# Autodesk Inventor assembly: sense3
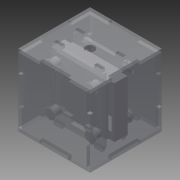
[picture p0: Inventor's stored thumbnail of the model, 180x180]
Saved by Autodesk Inventor 2013 (Build 170138000, 138)
## iProperties
Created: 2014-05-23
Part Number: sense3
Document SubType Name: Assembly
Designer: balogh
Author: balogh
## Documents named in this file (9)
- C:\Users\Brett Ian Balogh\Documents\GitHub\sense_cube\sense3_inventor\sense3.iam
- C:\Users\Brett Ian Balogh\Documents\GitHub\sense_cube\sense3_inventor\inside_box_top_bot.ipt
- C:\Users\Brett Ian Balogh\Documents\GitHub\sense_cube\sense3_inventor\pcb_mount.ipt
- C:\Users\Brett Ian Balogh\Documents\GitHub\sense_cube\sense3_inventor\battery_mount.ipt
- C:\Users\Brett Ian Balogh\Documents\GitHub\sense_cube\sense3_inventor\pcb.ipt
- C:\Users\Brett Ian Balogh\Documents\GitHub\sense_cube\sense3_inventor\inside_box_front_back.ipt
- C:\Users\Brett Ian Balogh\Documents\GitHub\sense_cube\sense3_inventor\inside_box_left_right.ipt
- C:\Users\Brett Ian Balogh\Documents\GitHub\sense_cube\sense3_inventor\thumbscrew_6-32x1.ipt
- C:\Users\Brett Ian Balogh\Documents\GitHub\sense_cube\sense3_inventor\thumbnut_6-32.ipt
## Components (22 placed, 8 different names)
1. inside_box_top_bot:1 — Angle:1, Mate:1, Mate:2, Mate:3, Mate:4, Flush:3, Flush:4, Mate:17, Mate:21, Mate:22
2. inside_box_top_bot:2 — Mate:5, Mate:6, Flush:1, Flush:2, Mate:13, Flush:5, Mate:14, Mate:15, Flush:6, Mate:16, Mate:20, Flush:7
3. pcb_mount:1 — Mate:3, Mate:4, Flush:2, Flush:4, Insert:21, Insert:22, Insert:23, Insert:24
4. pcb_mount:2 — Angle:1, Mate:1, Mate:2, Mate:5, Mate:6, Flush:1, Mate:12, Flush:3, Insert:17, Insert:18, Insert:19, Insert:20
5. battery_mount:1 — Insert:7, Insert:8, Insert:9, Insert:10
6. battery_mount:2 — Insert:9, Insert:10, Insert:11, Insert:12
7. battery_mount:3 — Insert:11, Insert:12, Insert:13, Insert:14
8. battery_mount:4 — Insert:13, Insert:14, Insert:15, Insert:16
9. pcb:1 — Insert:15, Insert:16
10. pcb:2 — Insert:7, Insert:8, Mate:12
11. inside_box_front_back:1 — Mate:13, Flush:5, Mate:14, Mate:18, Mate:19
12. inside_box_front_back:2 — Mate:15, Flush:6, Mate:16
13. inside_box_left_right:1 — Mate:17, Mate:18, Mate:19
14. inside_box_left_right:2 — Mate:20, Mate:21, Mate:22, Flush:7
15. thumbscrew_6-32x1:1 — Insert:18
16. thumbscrew_6-32x1:2 — Insert:19
17. thumbscrew_6-32x1:3 — Insert:20
18. thumbscrew_6-32x1:4 — Insert:17
19. thumbnut_6-32:1 — Insert:24
20. thumbnut_6-32:2 — Insert:22
21. thumbnut_6-32:3 — Insert:21
22. thumbnut_6-32:4 — Insert:23
## Relationships (43: Insert 18, Mate 17, Flush 7, Angle 1)
- Angle:1 (0 deg): inside_box_top_bot:1 ↔ pcb_mount:2
- Mate:1: inside_box_top_bot:1 ↔ pcb_mount:2
- Mate:2: inside_box_top_bot:1 ↔ pcb_mount:2
- Mate:3: inside_box_top_bot:1 ↔ pcb_mount:1
- Mate:4: inside_box_top_bot:1 ↔ pcb_mount:1
- Mate:5: inside_box_top_bot:2 ↔ pcb_mount:2
- Mate:6: inside_box_top_bot:2 ↔ pcb_mount:2
- Flush:1: inside_box_top_bot:2 ↔ pcb_mount:2
- Insert:7: battery_mount:1 ↔ pcb:2
- Insert:8: battery_mount:1 ↔ pcb:2
- Mate:12: pcb_mount:2 ↔ pcb:2
- Insert:9: battery_mount:1 ↔ battery_mount:2
- Insert:10: battery_mount:1 ↔ battery_mount:2
- Insert:11: battery_mount:2 ↔ battery_mount:3
- Insert:12: battery_mount:2 ↔ battery_mount:3
- Insert:13: battery_mount:3 ↔ battery_mount:4
- Insert:14: battery_mount:3 ↔ battery_mount:4
- Insert:15: battery_mount:4 ↔ pcb:1
- Insert:16: battery_mount:4 ↔ pcb:1
- Flush:2: inside_box_top_bot:2 ↔ pcb_mount:1
- Flush:3: inside_box_top_bot:1 ↔ pcb_mount:2
- Flush:4: inside_box_top_bot:1 ↔ pcb_mount:1
- Mate:13: inside_box_top_bot:2 ↔ inside_box_front_back:1
- Flush:5: inside_box_top_bot:2 ↔ inside_box_front_back:1
- Mate:14: inside_box_top_bot:2 ↔ inside_box_front_back:1
- Mate:15: inside_box_top_bot:2 ↔ inside_box_front_back:2
- Flush:6: inside_box_top_bot:2 ↔ inside_box_front_back:2
- Mate:16: inside_box_top_bot:2 ↔ inside_box_front_back:2
- Mate:17: inside_box_top_bot:1 ↔ inside_box_left_right:1
- Mate:18: inside_box_front_back:1 ↔ inside_box_left_right:1
- Mate:19: inside_box_front_back:1 ↔ inside_box_left_right:1
- Mate:20: inside_box_top_bot:2 ↔ inside_box_left_right:2
- Mate:21: inside_box_top_bot:1 ↔ inside_box_left_right:2
- Mate:22: inside_box_top_bot:1 ↔ inside_box_left_right:2
- Flush:7: inside_box_top_bot:2 ↔ inside_box_left_right:2
- Insert:17: pcb_mount:2 ↔ thumbscrew_6-32x1:4
- Insert:18: pcb_mount:2 ↔ thumbscrew_6-32x1:1
- Insert:19: pcb_mount:2 ↔ thumbscrew_6-32x1:2
- Insert:20: pcb_mount:2 ↔ thumbscrew_6-32x1:3
- Insert:21: pcb_mount:1 ↔ thumbnut_6-32:3
- Insert:22: pcb_mount:1 ↔ thumbnut_6-32:2
- Insert:23: pcb_mount:1 ↔ thumbnut_6-32:4
- Insert:24: pcb_mount:1 ↔ thumbnut_6-32:1
